# Autodesk Inventor assembly: Assembly1
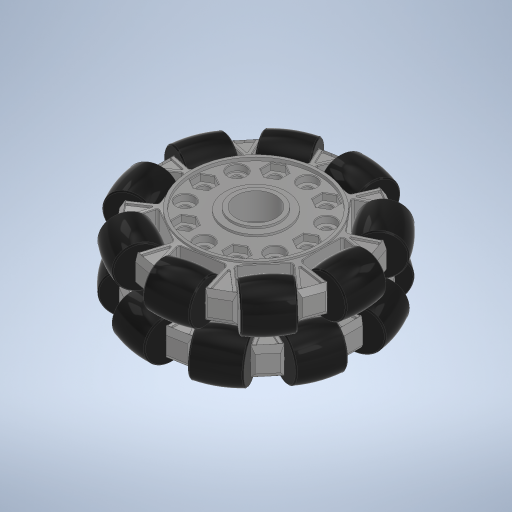
[picture p0: Inventor's stored thumbnail of the model, 512x512]
Saved by Autodesk Inventor 2024 (Build 280153000, 153)
## iProperties
Created: 2023-12-18
Part Number: Assembly1
Document SubType Name: Assembly
Designer: SAHITYA
Author: SAHITYA
## Documents named in this file (3)
- C:\Users\SAHITYA\OneDrive\Documents\Robotics\Assembly1.iam
- C:\Users\SAHITYA\OneDrive\Documents\Robotics\Part1.ipt
- C:\Users\SAHITYA\OneDrive\Documents\Robotics\Part2.ipt
## Components (21 placed, 2 different names)
1. Part1:1 — Mate:2, Mate:3, Mate:4, Mate:5, Mate:6, Mate:9
2. Part1:2 — Mate:2, Mate:3, Mate:7, Mate:8, Mate:9
3. Part2:1 — Mate:4, Mate:5, Mate:6
4. Part2:2
5. Part2:3
6. Part2:4
7. Part2:5
8. Part2:6
9. Part2:7
10. Part2:8
11. Part2:9
12. Part2:10
13. Part2:11 — Mate:7, Mate:8
14. Part2:12
15. Part2:13
16. Part2:14
17. Part2:15
18. Part2:16
19. Part2:17
20. Part2:18
21. Part2:19
## Component patterns: (10 elements, first: Part2:1), (9 elements, first: Part2:11)
## Relationships (8: Mate 8)
- Mate:2: Part1:1 ↔ Part1:2
- Mate:3: Part1:1 ↔ Part1:2
- Mate:4: Part1:1 ↔ Part2:1
- Mate:5: Part1:1 ↔ Part2:1
- Mate:6 (0.3 mm): Part1:1 ↔ Part2:1
- Mate:7: Part1:2 ↔ Part2:11
- Mate:8 (0.3 mm): Part1:2 ↔ Part2:11
- Mate:9: Part1:1 ↔ Part1:2
